# Autodesk Inventor assembly: ASY NDM-VOS_powder_hopper
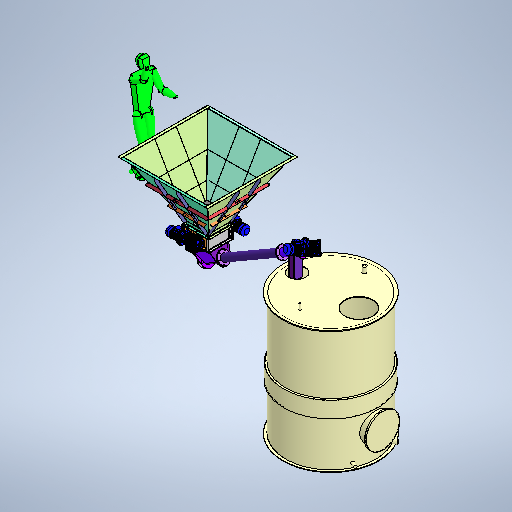
[picture p0: Inventor's stored thumbnail of the model, 512x512]
Saved by Autodesk Inventor 2025 (Build 290162010, 162A)
## iProperties
Created: 2024-07-24
Part Number: ASY NDM-VOS_powder_hopper
Document SubType Name: Assembly
Designer: admin
Author: admin
## Documents named in this file (18)
- C:\Users\admin\YandexDisk-badmisterfox\домашниий пк\Inventor\NDM-VOS_powder_hopper\ASY NDM-VOS_powder_hopper.iam
- C:\Users\admin\YandexDisk-badmisterfox\домашниий пк\Inventor\NDM-VOS_powder_hopper\human 01\ч ASY human dummy 01.iam
- C:\Users\admin\YandexDisk-badmisterfox\домашниий пк\Inventor\NDM-VOS_powder_hopper\NDM-VOS dummy3.ipt
- C:\Users\admin\YandexDisk-badmisterfox\домашниий пк\Inventor\NDM-VOS_powder_hopper\NDM-VOS dummy5.ipt
- C:\Users\admin\YandexDisk-badmisterfox\домашниий пк\Inventor\NDM-VOS_powder_hopper\NDM-VOS dummy FLOOR.ipt
- C:\Users\admin\YandexDisk-badmisterfox\домашниий пк\Inventor\NDM-VOS_powder_hopper\NDM-VOS dummy Crane.ipt
- C:\Users\admin\YandexDisk-badmisterfox\домашниий пк\Inventor\NDM-VOS_powder_hopper\NDM-VOS dummy upstairse.ipt
- C:\Users\admin\YandexDisk-badmisterfox\домашниий пк\Inventor\NDM-VOS_powder_hopper\Workspaces\Workspace\Cone\ASY MSC 100 cone.iam
- C:\Users\admin\YandexDisk-badmisterfox\домашниий пк\Inventor\NDM-VOS_powder_hopper\ASY HPR 200  Frame.iam
- C:\Users\admin\YandexDisk-badmisterfox\домашниий пк\Inventor\NDM-VOS_powder_hopper\TM06198C pump.ipt
- C:\Users\admin\YandexDisk-badmisterfox\домашниий пк\Inventor\NDM-VOS_powder_hopper\ASY HPR 300 Frame human.iam
- C:\Users\admin\YandexDisk-badmisterfox\домашниий пк\Inventor\NDM-VOS_powder_hopper\ASY_Ступень.iam
- C:\Users\admin\YandexDisk-badmisterfox\домашниий пк\Inventor\NDM-VOS_powder_hopper\ASY стойка.iam
- C:\Users\admin\YandexDisk-badmisterfox\домашниий пк\Inventor\NDM-VOS_powder_hopper\ISO 4019 - 80x40x2 - 2500.ipt
- C:\Users\admin\YandexDisk-badmisterfox\домашниий пк\Inventor\NDM-VOS_powder_hopper\ASY NVPH-400 shredder.iam
- C:\Users\admin\YandexDisk-badmisterfox\домашниий пк\Inventor\Content Center Files\en-US\ISO 4775\ISO 4775 - M12.ipt
- C:\Users\admin\YandexDisk-badmisterfox\домашниий пк\Inventor\NDM-VOS_powder_hopper\3d party\PCRV080-075SHFA_MS80B5\PCRV080-075SHFA_MS80B5\PCRV080-075SHFA_MS80B5.ipt
- C:\Users\admin\YandexDisk-badmisterfox\домашниий пк\Inventor\NDM-VOS_powder_hopper\ASY NVPH-300 hopper.iam
## Components (37 placed, 17 different names)
1. NDM-VOS dummy3:1 — Mate:5, Mate:9
2. NDM-VOS dummy3:2 — Mate:6, Mate:8, Mate:9, Flush:15
3. NDM-VOS dummy5:1 — Mate:14, Flush:16
4. NDM-VOS dummy5:2 — Flush:9, Flush:15, Mate:14
5. ч ASY human dummy 01:1 [sub-assembly]
6. NDM-VOS dummy FLOOR:1 — Mate:5, Mate:6, Mate:8, Mate:10, Flush:16, Mate:18
7. NDM-VOS dummy Crane:1 — Mate:10
8. NDM-VOS dummy upstairse:1 — Mate:18, Mate:23
9. ASY MSC 100 CONE:1 [sub-assembly] — Flush:19, Mate:19, Mate:20, Rigid:27
10. ASY HPR 200  Frame:1 [sub-assembly] — Flush:19, Mate:19, Mate:20, Flush:20, Flush:21, Mate:21, Rigid:3
11. TM06198C pump:1
12. ASY HPR 300 Frame human:1 [sub-assembly]
13. ASY стойка:1 [sub-assembly] — Flush:20, Flush:21, Mate:21, Flush:22, Flush:23, Mate:22, Rigid:5, Rigid:6
14. ASY HPR 200  Frame:2 [sub-assembly] — Flush:22, Flush:23, Mate:22, Mate:26
15. ASY стойка:2 [sub-assembly] — Rigid:3, Rigid:4
16. ASY стойка:3 [sub-assembly] — Rigid:4, Flush:25
17. ISO 4019 - 80x40x2 - 2700:1 — Rigid:5
18. ISO 4019 - 80x40x2 - 2700:2
19. ISO 4019 - 80x40x2 - 2700:3 — Rigid:6, Flush:24, Mate:24
20. ASY MSC 100 CONE:2 [sub-assembly] — Mate:26
21. TM06198C pump:2
22. ASY NVPH-400 shredder:1 [sub-assembly] — Rigid:27, Mate:31, Mate:32
23. ISO 4775 M12:1 — Mate:31, Mate:32
24. PCRV080-075SHFA_MS80B5:1
25. ASY NVPH-300 hopper:1 [sub-assembly]
26. ASY_Ступень:1 [sub-assembly] — Flush:24, Mate:23, Mate:24, Flush:25
27. ASY_Ступень:2 [sub-assembly]
28. ASY_Ступень:3 [sub-assembly]
29. ASY_Ступень:4 [sub-assembly]
30. ASY_Ступень:5 [sub-assembly]
31. ASY_Ступень:6 [sub-assembly]
32. ASY_Ступень:7 [sub-assembly]
33. ASY_Ступень:8 [sub-assembly]
34. ASY_Ступень:9 [sub-assembly]
35. ASY_Ступень:10 [sub-assembly]
36. ASY_Ступень:11 [sub-assembly]
37. ASY_Ступень:12 [sub-assembly]
## Component patterns: (12 elements, first: ASY_Ступень:1)
## Relationships (38: Mate 19, Flush 12, WeldJoint 6, RevoluteJoint 1)
- Flush:9: NDM-VOS dummy5:2
- Mate:5: NDM-VOS dummy3:1 ↔ NDM-VOS dummy FLOOR:1
- Mate:6: NDM-VOS dummy3:2 ↔ NDM-VOS dummy FLOOR:1
- Mate:8 (1200 mm): NDM-VOS dummy3:2 ↔ NDM-VOS dummy FLOOR:1
- Mate:9 (-1830 mm): NDM-VOS dummy3:1 ↔ NDM-VOS dummy3:2
- Mate:10 (3500 mm): NDM-VOS dummy FLOOR:1 ↔ NDM-VOS dummy Crane:1
- [Mate]: NDM-VOS dummy3:2 ↔ ASY MSC 100 CONE:1
- Flush:15: NDM-VOS dummy3:2 ↔ NDM-VOS dummy5:2
- Mate:14: NDM-VOS dummy5:1 ↔ NDM-VOS dummy5:2
- Flush:16: NDM-VOS dummy5:1 ↔ NDM-VOS dummy FLOOR:1
- Mate:18: NDM-VOS dummy FLOOR:1 ↔ NDM-VOS dummy upstairse:1
- [Flush]: ASY HPR 200  Frame:1
- Flush:19: ASY MSC 100 CONE:1 ↔ ASY HPR 200  Frame:1
- Mate:19: ASY MSC 100 CONE:1 ↔ ASY HPR 200  Frame:1
- Mate:20: ASY MSC 100 CONE:1 ↔ ASY HPR 200  Frame:1
- Flush:20: ASY HPR 200  Frame:1 ↔ ASY стойка:1
- Flush:21: ASY HPR 200  Frame:1 ↔ ASY стойка:1
- Mate:21: ASY HPR 200  Frame:1 ↔ ASY стойка:1
- Flush:22: ASY стойка:1 ↔ ASY HPR 200  Frame:2
- Flush:23: ASY стойка:1 ↔ ASY HPR 200  Frame:2
- Mate:22: ASY стойка:1 ↔ ASY HPR 200  Frame:2
- Rigid:3 [WeldJoint]: ASY HPR 200  Frame:1 ↔ ASY стойка:2
- Rigid:4 [WeldJoint] (1000 mm): ASY стойка:2 ↔ ASY стойка:3
- Rigid:5 [WeldJoint]: ASY стойка:1 ↔ ISO 4019 - 80x40x2 - 2700:1
- Rigid:6 [WeldJoint]: ASY стойка:1 ↔ ISO 4019 - 80x40x2 - 2700:3
- Flush:24 (182 mm): ISO 4019 - 80x40x2 - 2700:3 ↔ ASY_Ступень:1
- Mate:23: NDM-VOS dummy upstairse:1 ↔ ASY_Ступень:1
- Mate:24: ISO 4019 - 80x40x2 - 2700:3 ↔ ASY_Ступень:1
- Flush:25: ASY стойка:3 ↔ ASY_Ступень:1
- Mate:26: ASY HPR 200  Frame:2 ↔ ASY MSC 100 CONE:2
- Rigid:27 [WeldJoint]: ASY MSC 100 CONE:1 ↔ ASY NVPH-400 shredder:1
- [WeldJoint]: ASY NVPH-400 shredder:1 ↔ ASY NVPH-300 hopper:1
- [Mate]: ASY NVPH-400 shredder:1 ↔ ASY NVPH-300 hopper:1
- [Flush]: ASY NVPH-400 shredder:1 ↔ ASY NVPH-300 hopper:1
- Mate:31: ASY NVPH-400 shredder:1 ↔ ISO 4775 M12:1
- Mate:32: ASY NVPH-400 shredder:1 ↔ ISO 4775 M12:1
- [RevoluteJoint] (100 mm): PCRV080-075SHFA_MS80B5:1 ↔ ASY NVPH-300 hopper:1
- [Mate]: ASY NVPH-400 shredder:1 ↔ ASY NVPH-300 hopper:1
